# Autodesk Inventor assembly: servo motor HS-7955TG
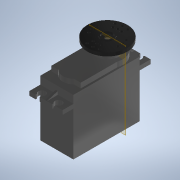
[picture p0: Inventor's stored thumbnail of the model, 180x180]
Saved by Autodesk Inventor 2022.6 (Build 266554000, 554)
## iProperties
Created: 2017-12-19
Part Number: servo motor HS-7955TG
Document SubType Name: Assembly
Designer: s41607
Author: s41607
## Documents named in this file (3)
- C:\Users\Zhong\Desktop\SP\YR_3_SEM_1\WRO\Robot\vehicle v4.6\vehicle v4.6\servo motor HS-7955TG.iam
- C:\Users\Zhong\Desktop\SP\YR_3_SEM_1\WRO\Robot\vehicle v4.6\vehicle v4.6\servo motor HS-7955TG.ipt
- C:\Users\Zhong\Desktop\SP\YR_3_SEM_1\WRO\Robot\vehicle v4.6\vehicle v4.6\servo motor HS-7955TG round horn.ipt
## Components (2 placed, 2 different names)
1. servo motor HS-7955TG:1 — Flush:1, Flush:2, Flush:3, Insert:1, Flush:4
2. servo motor HS-7955TG round horn:1 — Insert:1
## Relationships (5: Flush 4, Insert 1)
- Flush:1: servo motor HS-7955TG:1
- Flush:2: servo motor HS-7955TG:1
- Flush:3: servo motor HS-7955TG:1
- Insert:1: servo motor HS-7955TG:1 ↔ servo motor HS-7955TG round horn:1
- Flush:4 (-30.5 mm): servo motor HS-7955TG:1
